# Autodesk Inventor assembly: panel
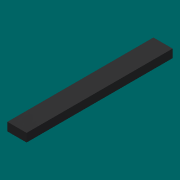
[picture p0: Inventor's stored thumbnail of the model, 180x180]
Saved by Autodesk Inventor 2016 (Build 200138000, 138)
## iProperties
Created: 2016-02-15
Part Number: panel
Document SubType Name: Assembly
Designer: sawai
Author: sawai
## Documents named in this file (4)
- C:\Users\Sawaiz\OneDrive\projects\scintillatorPanel\panel.iam
- C:\Users\Sawaiz\OneDrive\projects\scintillatorPanel\rawPanel.iam
- C:\Users\Sawaiz\OneDrive\projects\scintillatorPanel\rubberizedCoating.ipt
- C:\Users\Sawaiz\OneDrive\projects\scintillatorPanel\silvering.ipt
## Components (3 placed, 3 different names)
1. rawPanel:1 [sub-assembly] — Mate:3, Mate:4, Flush:2
2. rubberizedCoating:1 — Mate:1, Mate:2, Flush:1, Flush:2
3. silvering:1 — Mate:1, Mate:2, Flush:1, Mate:3, Mate:4
## Relationships (6: Mate 4, Flush 2)
- Mate:1: rubberizedCoating:1 ↔ silvering:1
- Mate:2: rubberizedCoating:1 ↔ silvering:1
- Flush:1: rubberizedCoating:1 ↔ silvering:1
- Mate:3: rawPanel:1 ↔ silvering:1
- Mate:4: rawPanel:1 ↔ silvering:1
- Flush:2: rawPanel:1 ↔ rubberizedCoating:1
